# Autodesk Inventor assembly: 全体v1
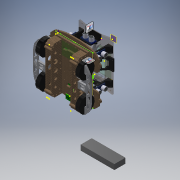
[picture p0: Inventor's stored thumbnail of the model, 180x180]
Saved by Autodesk Inventor 2018 (Build 220112000, 112)
## iProperties
Created: 2018-11-27
Part Number: 全体v1
Material: 一般
Document SubType Name: Assembly
Designer: shun2
Author: shun2
## Documents named in this file (22)
- C:\Users\rakur\Documents\Aquila-drawings-2018-\全体v1.iam
- C:\Users\rakur\Documents\Aquila-drawings-2018-\ギアボックス\ギアボックスv2.iam
- C:\Users\rakur\Documents\Aquila-drawings-2018-\1枚目\一枚目.ipt
- C:\Users\rakur\Documents\Aquila-drawings-2018-\基板保護2018.8.7.ipt
- C:\Users\rakur\Documents\Aquila-drawings-2018-\2枚目\2枚目.ipt
- C:\Users\rakur\Documents\Aquila-drawings-2018-\3枚目\3枚目v4.ipt
- C:\Users\rakur\Documents\Aquila-drawings-2018-\ping-module.iam
- C:\Users\rakur\Documents\Aquila-drawings-2018-\pingmodule-y.iam
- C:\Users\rakur\Documents\Aquila-drawings-2018-\OpenMVMount-Tate.iam
- C:\Users\rakur\Documents\Aquila-drawings-2018-\Color.ipt
- C:\Users\rakur\Documents\Aquila-drawings-2018-\モタドラ.ipt
- C:\Users\rakur\Documents\Aquila-drawings-2018-\メイン基板.ipt
- C:\Users\rakur\Documents\Aquila-drawings-2018-\Aquila-2018-Under.ipt
- C:\Users\rakur\Documents\Aquila-drawings-2018-\LiFePo.ipt
- C:\Users\rakur\Documents\Aquila-drawings-2018-\LiFeGuard.ipt
- C:\Users\rakur\Documents\Aquila-drawings-2018-\Ping-front.ipt
- C:\Users\rakur\Documents\Aquila-drawings-2018-\Tire.ipt
- C:\Users\rakur\Documents\Aquila-drawings-2018-\ガイド\ガイド横v1.ipt
- C:\Users\rakur\Documents\Aquila-drawings-2018-\レスキューキット投下機構\RescueKit-Pipev3.ipt
- C:\Users\rakur\Documents\Aquila-drawings-2018-\レスキューキット投下機構\RescueKit-Slidev2.ipt
- C:\Users\rakur\Documents\Aquila-drawings-2018-\レスキューキット投下機構\28BYJ-48.ipt
- C:\Users\rakur\Documents\Aquila-drawings-2018-\レスキューキット投下機構\RescueKit-Gear-18.ipt
## Components (31 placed, 21 different names)
1. 一枚目:1 — メイト:1, メイト:2, フラッシュ:1, フラッシュ:2, フラッシュ:3, フラッシュ:4, メイト:3, メイト:4, メイト:5, メイト:44, メイト:45, メイト:46, メイト:47, メイト:48, メイト:49, メイト:53, メイト:54, メイト:55, メイト:95, メイト:151
2. 2枚目:1 — メイト:6, メイト:7, メイト:8, メイト:41, メイト:42, メイト:74, メイト:75, メイト:76, メイト:94, メイト:105, メイト:106, メイト:107, メイト:108, メイト:109, メイト:110, メイト:111, メイト:112, メイト:113, メイト:127, メイト:157
3. 3枚目v4:1 — メイト:41, メイト:42, メイト:50, メイト:51, メイト:52, メイト:94, メイト:121, メイト:122, メイト:123, メイト:124, メイト:125, メイト:126, メイト:127, メイト:132, メイト:133, メイト:134, メイト:135, メイト:136, メイト:137, メイト:138, メイト:139, メイト:140, メイト:141, メイト:142, メイト:143, メイト:144, メイト:145, メイト:146, メイト:147, メイト:148, メイト:149, メイト:154, メイト:155, メイト:156
4. 基板保護2018.8.7:1 — メイト:3, メイト:4, メイト:5, メイト:6, メイト:7, メイト:8
5. LiFePo:1
6. LiFeGuard:2 — メイト:108, メイト:109, メイト:110
7. ガイド横v1:1 — メイト:105, メイト:106, メイト:107
8. ガイド横v1:2 — メイト:111, メイト:112, メイト:113
9. RescueKit-Pipev3:1 — メイト:154, メイト:155, メイト:156, フラッシュ:5, フラッシュ:6, フラッシュ:7
10. RescueKit-Slidev2:1 — メイト:157, フラッシュ:5
11. 28BYJ-48:1 — フラッシュ:6, フラッシュ:7
12. RescueKit-Gear-18:1
13. Ping-front:1 — メイト:74, メイト:75, メイト:76
14. ping-module:1 [sub-assembly] — メイト:132, メイト:133, メイト:134
15. ping-module:2 [sub-assembly] — メイト:141, メイト:142, メイト:143
16. ping-module:3 [sub-assembly] — メイト:138, メイト:139, メイト:140
17. ping-module:4 [sub-assembly] — メイト:135, メイト:136, メイト:137
18. pingmodule-y:1 [sub-assembly] — メイト:144, メイト:145, メイト:146
19. OpenMVMount-Tate:1 [sub-assembly] — メイト:121, メイト:122, メイト:126
20. OpenMVMount-Tate:2 [sub-assembly] — メイト:123, メイト:124, メイト:125
21. OpenMVMount-Tate:3 [sub-assembly] — メイト:147, メイト:148, メイト:149
22. Color:1 — メイト:44, メイト:45, メイト:46
23. モタドラ:1 — メイト:47, メイト:48, メイト:49
24. メイン基板:1 — メイト:50, メイト:51, メイト:52
25. Aquila-2018-Under:2 — メイト:53, メイト:54, メイト:55
26. Tire:1 — メイト:86, メイト:87
27. Tire:2 — メイト:88, メイト:89
28. Tire:3 — メイト:92, メイト:93
29. Tire:4 — メイト:90, メイト:91
30. ギアボックスv2:2 [sub-assembly] — メイト:2, フラッシュ:1, フラッシュ:4, メイト:86, メイト:87, メイト:88, メイト:89
31. ギアボックスv2:1 [sub-assembly] — メイト:1, フラッシュ:2, フラッシュ:3, メイト:90, メイト:91, メイト:92, メイト:93, メイト:96
## Relationships (82: Mate 75, Flush 7)
- メイト:1 [Mate] (3 mm): 一枚目:1 ↔ ギアボックスv2:1
- メイト:2 [Mate] (3 mm): 一枚目:1 ↔ ギアボックスv2:2
- フラッシュ:1 [Flush]: 一枚目:1 ↔ ギアボックスv2:2
- フラッシュ:2 [Flush]: 一枚目:1 ↔ ギアボックスv2:1
- フラッシュ:3 [Flush] (2 mm): 一枚目:1 ↔ ギアボックスv2:1
- フラッシュ:4 [Flush] (2 mm): 一枚目:1 ↔ ギアボックスv2:2
- メイト:3 [Mate] (0.2 mm): 一枚目:1 ↔ 基板保護2018.8.7:1
- メイト:4 [Mate]: 一枚目:1 ↔ 基板保護2018.8.7:1
- メイト:5 [Mate]: 一枚目:1 ↔ 基板保護2018.8.7:1
- メイト:6 [Mate] (3 mm): 2枚目:1 ↔ 基板保護2018.8.7:1
- メイト:7 [Mate]: 2枚目:1 ↔ 基板保護2018.8.7:1
- メイト:8 [Mate]: 2枚目:1 ↔ 基板保護2018.8.7:1
- メイト:41 [Mate] (80 mm): 2枚目:1 ↔ 3枚目v4:1
- メイト:42 [Mate]: 2枚目:1 ↔ 3枚目v4:1
- メイト:44 [Mate] (40 mm): 一枚目:1 ↔ Color:1
- メイト:45 [Mate]: 一枚目:1 ↔ Color:1
- メイト:46 [Mate]: 一枚目:1 ↔ Color:1
- メイト:47 [Mate] (8 mm): 一枚目:1 ↔ モタドラ:1
- メイト:48 [Mate]: 一枚目:1 ↔ モタドラ:1
- メイト:49 [Mate]: 一枚目:1 ↔ モタドラ:1
- メイト:50 [Mate] (8 mm): 3枚目v4:1 ↔ メイン基板:1
- メイト:51 [Mate]: 3枚目v4:1 ↔ メイン基板:1
- メイト:52 [Mate]: 3枚目v4:1 ↔ メイン基板:1
- メイト:53 [Mate] (3 mm): 一枚目:1 ↔ Aquila-2018-Under:2
- メイト:54 [Mate]: 一枚目:1 ↔ Aquila-2018-Under:2
- メイト:55 [Mate]: 一枚目:1 ↔ Aquila-2018-Under:2
- メイト:74 [Mate]: 2枚目:1 ↔ Ping-front:1
- メイト:75 [Mate]: 2枚目:1 ↔ Ping-front:1
- メイト:76 [Mate]: 2枚目:1 ↔ Ping-front:1
- メイト:86 [Mate] (8 mm): Tire:1 ↔ ギアボックスv2:2
- メイト:87 [Mate]: Tire:1 ↔ ギアボックスv2:2
- メイト:88 [Mate] (8 mm): Tire:2 ↔ ギアボックスv2:2
- メイト:89 [Mate]: Tire:2 ↔ ギアボックスv2:2
- メイト:90 [Mate]: Tire:4 ↔ ギアボックスv2:1
- メイト:91 [Mate] (8 mm): Tire:4 ↔ ギアボックスv2:1
- メイト:92 [Mate]: Tire:3 ↔ ギアボックスv2:1
- メイト:93 [Mate] (8 mm): Tire:3 ↔ ギアボックスv2:1
- メイト:94 [Mate]: 2枚目:1 ↔ 3枚目v4:1
- メイト:95 [Mate]: 一枚目:1
- メイト:96 [Mate]: ギアボックスv2:1
- メイト:105 [Mate] (45 mm): 2枚目:1 ↔ ガイド横v1:1
- メイト:106 [Mate]: 2枚目:1 ↔ ガイド横v1:1
- メイト:107 [Mate]: 2枚目:1 ↔ ガイド横v1:1
- メイト:108 [Mate]: 2枚目:1 ↔ LiFeGuard:2
- メイト:109 [Mate]: 2枚目:1 ↔ LiFeGuard:2
- メイト:110 [Mate]: 2枚目:1 ↔ LiFeGuard:2
- メイト:111 [Mate] (45 mm): 2枚目:1 ↔ ガイド横v1:2
- メイト:112 [Mate]: 2枚目:1 ↔ ガイド横v1:2
- メイト:113 [Mate]: 2枚目:1 ↔ ガイド横v1:2
- メイト:121 [Mate]: 3枚目v4:1 ↔ OpenMVMount-Tate:1
- メイト:122 [Mate]: 3枚目v4:1 ↔ OpenMVMount-Tate:1
- メイト:123 [Mate]: 3枚目v4:1 ↔ OpenMVMount-Tate:2
- メイト:124 [Mate]: 3枚目v4:1 ↔ OpenMVMount-Tate:2
- メイト:125 [Mate]: 3枚目v4:1 ↔ OpenMVMount-Tate:2
- メイト:126 [Mate]: 3枚目v4:1 ↔ OpenMVMount-Tate:1
- メイト:127 [Mate]: 2枚目:1 ↔ 3枚目v4:1
- メイト:132 [Mate]: 3枚目v4:1 ↔ ping-module:1
- メイト:133 [Mate]: 3枚目v4:1 ↔ ping-module:1
- メイト:134 [Mate]: 3枚目v4:1 ↔ ping-module:1
- メイト:135 [Mate]: 3枚目v4:1 ↔ ping-module:4
- メイト:136 [Mate]: 3枚目v4:1 ↔ ping-module:4
- メイト:137 [Mate]: 3枚目v4:1 ↔ ping-module:4
- メイト:138 [Mate]: 3枚目v4:1 ↔ ping-module:3
- メイト:139 [Mate]: 3枚目v4:1 ↔ ping-module:3
- メイト:140 [Mate]: 3枚目v4:1 ↔ ping-module:3
- メイト:141 [Mate]: 3枚目v4:1 ↔ ping-module:2
- メイト:142 [Mate]: 3枚目v4:1 ↔ ping-module:2
- メイト:143 [Mate]: 3枚目v4:1 ↔ ping-module:2
- メイト:144 [Mate]: 3枚目v4:1 ↔ pingmodule-y:1
- メイト:145 [Mate]: 3枚目v4:1 ↔ pingmodule-y:1
- メイト:146 [Mate]: 3枚目v4:1 ↔ pingmodule-y:1
- メイト:147 [Mate]: 3枚目v4:1 ↔ OpenMVMount-Tate:3
- メイト:148 [Mate]: 3枚目v4:1 ↔ OpenMVMount-Tate:3
- メイト:149 [Mate]: 3枚目v4:1 ↔ OpenMVMount-Tate:3
- メイト:151 [Mate]: 一枚目:1
- メイト:154 [Mate]: 3枚目v4:1 ↔ RescueKit-Pipev3:1
- メイト:155 [Mate]: 3枚目v4:1 ↔ RescueKit-Pipev3:1
- メイト:156 [Mate]: 3枚目v4:1 ↔ RescueKit-Pipev3:1
- メイト:157 [Mate]: 2枚目:1 ↔ RescueKit-Slidev2:1
- フラッシュ:5 [Flush]: RescueKit-Pipev3:1 ↔ RescueKit-Slidev2:1
- フラッシュ:6 [Flush] (42 mm): RescueKit-Pipev3:1 ↔ 28BYJ-48:1
- フラッシュ:7 [Flush] (-7.75 mm): RescueKit-Pipev3:1 ↔ 28BYJ-48:1
